# Autodesk Inventor assembly: LegEncoderBoard
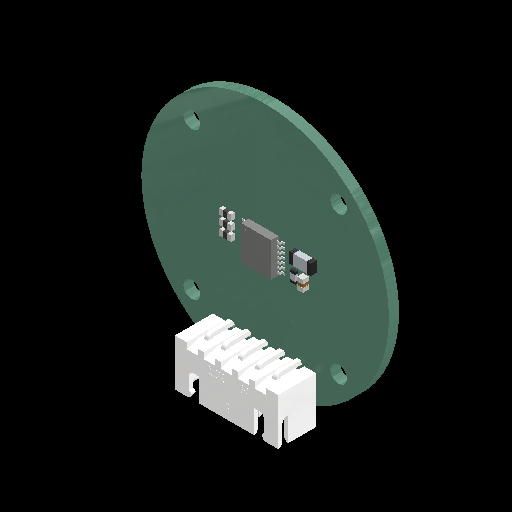
[picture p0: Inventor's stored thumbnail of the model, 512x512]
Saved by Autodesk Inventor 2025.2 (Build 292293000, 293)
## iProperties
Company: Kicad
Created: 2026-02-04
Part Number: LegEncoderBoard
Description: KiCad electronic assembly
Document SubType Name: Assembly
Designer: valer
Authority: Unknown
Sending System: KiCad to STEP converter
Preprocessor: Open CASCADE STEP processor 7.8
Title: LegEncoderBoard.step
Author: Pcbnew
## Documents named in this file (8)
- C:\Users\valer\Desktop\str1ker\cad\external\WheelEncoder\LegEncoderBoard.iam
- C:\Users\valer\Desktop\str1ker\cad\external\WheelEncoder\CC0603JRX7R7BB105.ipt
- C:\Users\valer\Desktop\str1ker\cad\external\WheelEncoder\CR0603-FX-4701ELF.ipt
- C:\Users\valer\Desktop\str1ker\cad\external\WheelEncoder\885012206089.iam
- C:\Users\valer\Desktop\str1ker\cad\external\WheelEncoder\TSSOP-14_AMS.ipt
- C:\Users\valer\Desktop\str1ker\cad\external\WheelEncoder\885342208002.iam
- C:\Users\valer\Desktop\str1ker\cad\external\WheelEncoder\LegEncoderBoard_PCB.ipt
- C:\Users\valer\Desktop\str1ker\cad\external\WheelEncoder\WHITE JST XH 5 PIN CONNECTOR - P 2.54mm - ANGLED.ipt
## Components (9 placed, 9 different names)
1. 1
2. 2
3. 6 [sub-assembly]
4. 7 — Flush:1, Mate:2
5. 11 [sub-assembly]
6. 13
7. 14
8. 15 — Mate:1
9. WHITE JST XH 5 PIN CONNECTOR - P 2.54mm - ANGLED:1 — Mate:1, Flush:1, Mate:2
## Relationships (3: Mate 2, Flush 1)
- Mate:1: 15 ↔ WHITE JST XH 5 PIN CONNECTOR - P 2.54mm - ANGLED:1
- Flush:1: 7 ↔ WHITE JST XH 5 PIN CONNECTOR - P 2.54mm - ANGLED:1
- Mate:2 (9.97 mm): 7 ↔ WHITE JST XH 5 PIN CONNECTOR - P 2.54mm - ANGLED:1
